# Autodesk Inventor assembly: Link_02_Assembly_V02
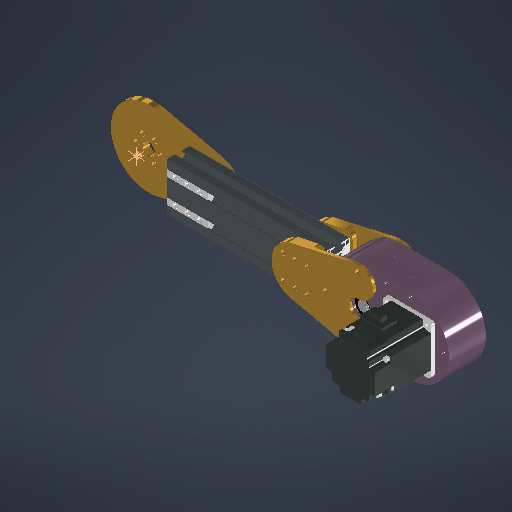
[picture p0: Inventor's stored thumbnail of the model, 512x512]
Saved by Autodesk Inventor 2026 (Build 300175000, 175)
## iProperties
Created: 2025-12-01
Part Number: Link_02_Assembly_V02
Document SubType Name: Assembly
Designer: DanielFGarzon
Mass: 2039.81 g
Surface Area: 3894.89 cm^2
Volume: 921.6 cm^3
Density: 2.21334 g/cm^3
Author: DanielFGarzon
## Documents named in this file (5)
- D:\POLIMI\3RD SEMESTER\Industrial Robotics\Project\Mine\Link_02_Assembly_V02.iam
- D:\POLIMI\3RD SEMESTER\Industrial Robotics\Project\Mine\Link_02.ipt
- D:\POLIMI\3RD SEMESTER\Industrial Robotics\Project\Mine\RotationalConector_30x60_V02.ipt
- D:\POLIMI\3RD SEMESTER\Industrial Robotics\Project\Mine\RigidConector_30x60.ipt
- D:\POLIMI\3RD SEMESTER\Industrial Robotics\Project\Mine\Reducer.iam
## Components (5 placed, 4 different names)
1. Link_02:1 — Mate:4, Mate:5, Mate:6, Mate:7, Mate:8, Mate:9, Mate:10, Mate:11, Mate:15, Mate:16, Flush:1
2. RotationalConector_30x60_V02:1 — Mate:3, Mate:4, Mate:5, Mate:15
3. RigidConector_30x60:1 — Mate:9, Mate:10, Mate:11, Mate:12, Mate:13, Mate:14
4. RigidConector_30x60:2 — Mate:6, Mate:7, Mate:8
5. Reducer:1 [sub-assembly] — Mate:12, Mate:13, Mate:14
## Relationships (15: Mate 14, Flush 1)
- Mate:3: RotationalConector_30x60_V02:1
- Mate:4: Link_02:1 ↔ RotationalConector_30x60_V02:1
- Mate:5: Link_02:1 ↔ RotationalConector_30x60_V02:1
- Mate:6: Link_02:1 ↔ RigidConector_30x60:2
- Mate:7: Link_02:1 ↔ RigidConector_30x60:2
- Mate:8: Link_02:1 ↔ RigidConector_30x60:2
- Mate:9: Link_02:1 ↔ RigidConector_30x60:1
- Mate:10: Link_02:1 ↔ RigidConector_30x60:1
- Mate:11: Link_02:1 ↔ RigidConector_30x60:1
- Mate:12: RigidConector_30x60:1 ↔ Reducer:1
- Mate:13: RigidConector_30x60:1 ↔ Reducer:1
- Mate:14: RigidConector_30x60:1 ↔ Reducer:1
- Mate:15: Link_02:1 ↔ RotationalConector_30x60_V02:1
- Mate:16: Link_02:1
- Flush:1: Link_02:1
